# Autodesk Inventor assembly: Platform Assembly
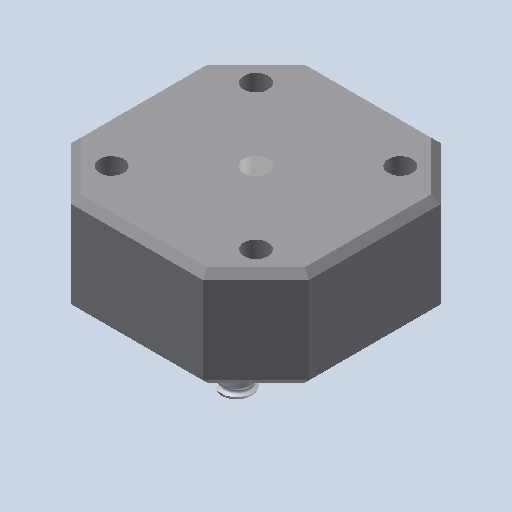
[picture p0: Inventor's stored thumbnail of the model, 512x512]
Saved by Autodesk Inventor 2025 (Build 290162000, 162)
## iProperties
Created: 2021-01-07
Part Number: Platform Assembly
Document SubType Name: Assembly
Designer: caleb
Author: caleb
## Documents named in this file (4)
- C:\Users\cfang\Desktop\nebraska-silicon-lab\Hardware\ETL\Module Assembly\Picker Tool - V2\Platform Assembly - V2.iam
- C:\Users\cfang\Desktop\nebraska-silicon-lab\Hardware\ETL\Module Assembly\Picker Tool - V2\Platform A - V2.ipt
- C:\Users\cfang\Desktop\nebraska-silicon-lab\Hardware\ETL\Module Assembly\Picker Tool - V2\Platform B - V2.ipt
- C:\Users\cfang\Desktop\nebraska-silicon-lab\Hardware\ETL\Module Assembly\Picker Tool - V2\3766A81_Extreme-Temperature Food Industry Vacuum Cup.ipt
## Components (5 placed, 3 different names)
1. Platform A - V2:1 — Mate:1, Flush:1, Flush:2
2. Platform B - V2:1 — Mate:1, Flush:1, Flush:2, Insert:2, Insert:4, Insert:5
3. 3766A81_Extreme-Temperature Food Industry Vacuum Cup:1 — Insert:2
4. 3766A81_Extreme-Temperature Food Industry Vacuum Cup:2 — Insert:5
5. 3766A81_Extreme-Temperature Food Industry Vacuum Cup:3 — Insert:4
## Relationships (6: Insert 3, Flush 2, Mate 1)
- Mate:1: Platform A - V2:1 ↔ Platform B - V2:1
- Flush:1: Platform A - V2:1 ↔ Platform B - V2:1
- Flush:2: Platform A - V2:1 ↔ Platform B - V2:1
- Insert:2: Platform B - V2:1 ↔ 3766A81_Extreme-Temperature Food Industry Vacuum Cup:1
- Insert:4: Platform B - V2:1 ↔ 3766A81_Extreme-Temperature Food Industry Vacuum Cup:3
- Insert:5: Platform B - V2:1 ↔ 3766A81_Extreme-Temperature Food Industry Vacuum Cup:2
